# Autodesk Inventor assembly: Box
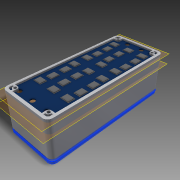
[picture p0: Inventor's stored thumbnail of the model, 180x180]
Saved by Autodesk Inventor 2016 (Build 200138000, 138)
## iProperties
Created: 2015-06-03
Part Number: Box
Document SubType Name: Assembly
Designer: Yann
plate_thickness: 3.000 mm
Author: Yann
## Documents named in this file (6)
- C:\Users\Yann\Documents\GitHub\BIKAIR_CAD\Source\Powertrain_Controller\Box.iam
- C:\Users\Yann\Documents\GitHub\BIKAIR_CAD\Source\Powertrain_Controller\Box_Bottom_Plate.ipt
- C:\Users\Yann\Documents\GitHub\BIKAIR_CAD\Source\Powertrain_Controller\Box_Top-Plate.ipt
- C:\Users\Yann\Documents\GitHub\BIKAIR_CAD\Source\Powertrain_Controller\Box_Body.ipt
- C:\Users\Yann\Documents\GitHub\BIKAIR_CAD\Source\Powertrain_Controller\Power_PCB.iam
- C:\Users\Yann\Documents\Inventor\Content Center Files\R2016\en-US\ANSI B18.6.5M(10)\ANSI B18.6.5M - M3x0.5 x 10(27).ipt
## Components (8 placed, 5 different names)
1. Box_Bottom_Plate:1 — Flush:1, Flush:2, Rigid:1, Rotational:1, Rotational:2, Rigid:2
2. Box_Top-Plate:1 — Flush:3, Flush:4, Flush:5
3. Box_Body:1 — Flush:6, Flush:7, Flush:8, Mate:2
4. Power_PCB:1 [sub-assembly] — Mate:1, Mate:2
5. Cross Recessed Flat Countersunk Head Tapping Screw - Type F - Type I - Metric M3x0.5 x 10:1 — Rigid:1
6. Cross Recessed Flat Countersunk Head Tapping Screw - Type F - Type I - Metric M3x0.5 x 10:2 — Rotational:2
7. Cross Recessed Flat Countersunk Head Tapping Screw - Type F - Type I - Metric M3x0.5 x 10:3 — Rotational:1
8. Cross Recessed Flat Countersunk Head Tapping Screw - Type F - Type I - Metric M3x0.5 x 10:4 — Rigid:2
## Relationships (14: Flush 8, Mate 2, WeldJoint 2, RevoluteJoint 2)
- Flush:1: Box_Bottom_Plate:1
- Flush:2: Box_Bottom_Plate:1
- Flush:3: Box_Top-Plate:1
- Flush:4: Box_Top-Plate:1
- Flush:5: Box_Top-Plate:1
- Flush:6: Box_Body:1
- Flush:7: Box_Body:1
- Flush:8: Box_Body:1
- Mate:1: Power_PCB:1
- Mate:2: Box_Body:1 ↔ Power_PCB:1
- Rigid:1 [WeldJoint]: Box_Bottom_Plate:1 ↔ Cross Recessed Flat Countersunk Head Tapping Screw - Type F - Type I - Metric M3x0.5 x 10:1
- Rotational:1 [RevoluteJoint]: Box_Bottom_Plate:1 ↔ Cross Recessed Flat Countersunk Head Tapping Screw - Type F - Type I - Metric M3x0.5 x 10:3
- Rotational:2 [RevoluteJoint]: Box_Bottom_Plate:1 ↔ Cross Recessed Flat Countersunk Head Tapping Screw - Type F - Type I - Metric M3x0.5 x 10:2
- Rigid:2 [WeldJoint]: Box_Bottom_Plate:1 ↔ Cross Recessed Flat Countersunk Head Tapping Screw - Type F - Type I - Metric M3x0.5 x 10:4
## Named parameters: plate_thickness = 3 mm
